# Autodesk Inventor assembly: правый привод_MIR
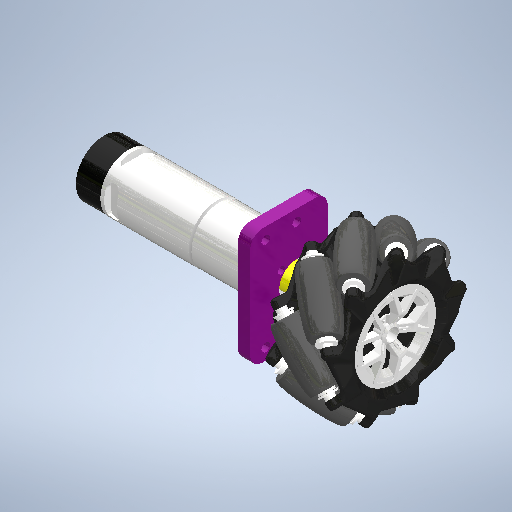
[picture p0: Inventor's stored thumbnail of the model, 512x512]
Saved by Autodesk Inventor 2025 (Build 290162000, 162)
## iProperties
Created: 2025-02-16
Part Number: правый привод_MIR
Document SubType Name: Assembly
Designer: volko
Author: volko
## Documents named in this file (5)
- C:\Users\volko\Desktop\диплом\diplom\Модели\детали\левый привод.iam
- C:\Users\volko\Desktop\диплом\diplom\Модели\детали\CHP-42GP-775 ABHL_MIR.ipt
- C:\Users\volko\Desktop\диплом\diplom\Модели\детали\кронштейн_MIR.ipt
- C:\Users\volko\Desktop\диплом\diplom\Модели\детали\переходная втулка_MIR.ipt
- C:\Users\volko\Desktop\диплом\diplom\Модели\Mecanum wheel - left\Mecanum wheel - left.iam
## Components (4 placed, 4 different names)
1. CHP-42GP-775 ABHL_MIR:1 — Совмещение:1, Совмещение:2, Заподлицо:1, Совмещение:3, Совмещение:4, Совмещение:5, Совмещение:11, Совмещение:12
2. кронштейн_MIR:1 — Совмещение:5, Совмещение:11, Совмещение:12
3. переходная втулка_MIR:1 — Совмещение:3, Совмещение:4, Совмещение:8, Совмещение:9, Совмещение:10, Заподлицо:18
4. Mecanum wheel - left:1 [sub-assembly] — Совмещение:8, Совмещение:9, Совмещение:10
## Relationships (12: Mate 10, Flush 2)
- Совмещение:1 [Mate]: CHP-42GP-775 ABHL_MIR:1
- Совмещение:2 [Mate]: CHP-42GP-775 ABHL_MIR:1
- Заподлицо:1 [Flush]: CHP-42GP-775 ABHL_MIR:1
- Совмещение:3 [Mate]: CHP-42GP-775 ABHL_MIR:1 ↔ переходная втулка_MIR:1
- Совмещение:4 [Mate]: CHP-42GP-775 ABHL_MIR:1 ↔ переходная втулка_MIR:1
- Совмещение:5 [Mate]: CHP-42GP-775 ABHL_MIR:1 ↔ кронштейн_MIR:1
- Совмещение:8 [Mate]: переходная втулка_MIR:1 ↔ Mecanum wheel - left:1
- Совмещение:9 [Mate]: переходная втулка_MIR:1 ↔ Mecanum wheel - left:1
- Совмещение:10 [Mate]: переходная втулка_MIR:1 ↔ Mecanum wheel - left:1
- Заподлицо:18 [Flush]: переходная втулка_MIR:1
- Совмещение:11 [Mate]: CHP-42GP-775 ABHL_MIR:1 ↔ кронштейн_MIR:1
- Совмещение:12 [Mate]: CHP-42GP-775 ABHL_MIR:1 ↔ кронштейн_MIR:1
